# Autodesk Inventor assembly: set1_to_print
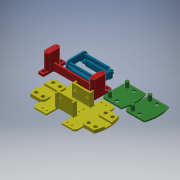
[picture p0: Inventor's stored thumbnail of the model, 180x180]
Saved by Autodesk Inventor 2017 SP1 (Build 210196100, 196)
## iProperties
Part Number: set1_to_print
Material: Générique
Document SubType Name: Assembly
Designer: tmonglon
Author: tmonglon
## Documents named in this file (5)
- D:\Inventor\Ahmet\ebug-chassis-june2017\retour fablab\design\set1_to_print.iam
- D:\Inventor\Ahmet\ebug-chassis-june2017\retour fablab\design\yellow_part.ipt
- D:\Inventor\Ahmet\ebug-chassis-june2017\retour fablab\design\blue_part.ipt
- D:\Inventor\Ahmet\ebug-chassis-june2017\retour fablab\design\green_part.ipt
- D:\Inventor\Ahmet\ebug-chassis-june2017\retour fablab\design\red_part.ipt
## Components (6 placed, 4 different names)
1. yellow_part:1 — Placage:1, Affleurement:1, Affleurement:2, Affleurement:3, Affleurement:4, Affleurement:5, Placage:4, Placage:5, Placage:7
2. blue_part:1 — Affleurement:5, Placage:2, Placage:3
3. blue_part:2 — Affleurement:4, Placage:2, Placage:3, Placage:6
4. green_part:1 — Affleurement:3, Affleurement:6, Placage:7
5. green_part:2 — Affleurement:2, Affleurement:6
6. red_part:1 — Affleurement:1, Placage:4, Placage:5, Placage:6
## Relationships (13: Mate 7, Flush 6)
- Placage:1 [Mate]: yellow_part:1
- Affleurement:1 [Flush]: yellow_part:1 ↔ red_part:1
- Affleurement:2 [Flush]: yellow_part:1 ↔ green_part:2
- Affleurement:3 [Flush]: yellow_part:1 ↔ green_part:1
- Affleurement:4 [Flush]: yellow_part:1 ↔ blue_part:2
- Affleurement:5 [Flush]: yellow_part:1 ↔ blue_part:1
- Placage:2 [Mate] (2 mm): blue_part:1 ↔ blue_part:2
- Placage:3 [Mate] (42 mm): blue_part:1 ↔ blue_part:2
- Placage:4 [Mate] (2 mm): yellow_part:1 ↔ red_part:1
- Placage:5 [Mate] (8 mm): yellow_part:1 ↔ red_part:1
- Placage:6 [Mate] (2 mm): blue_part:2 ↔ red_part:1
- Affleurement:6 [Flush]: green_part:1 ↔ green_part:2
- Placage:7 [Mate] (3 mm): yellow_part:1 ↔ green_part:1
